# Autodesk Inventor assembly: unitychan
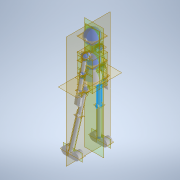
[picture p0: Inventor's stored thumbnail of the model, 180x180]
Saved by Autodesk Inventor 2021 (Build 250183000, 183)
## iProperties
Created: 2020-12-21
Part Number: unitychan
Document SubType Name: Assembly
Designer: Tazaki
Mass: 32000 g
Surface Area: 16434.1 cm^2
Volume: 27345.8 cm^3
Density: 1.1702 g/cm^3
Author: Tazaki
## Documents named in this file (19)
- C:\usr\Develop\choreonoid\BipedCnoid\model\unitychan\unitychan.iam
- C:\usr\Develop\choreonoid\BipedCnoid\model\unitychan\Hips.ipt
- C:\usr\Develop\choreonoid\BipedCnoid\model\unitychan\ChestY.ipt
- C:\usr\Develop\choreonoid\BipedCnoid\model\unitychan\ChestP.ipt
- C:\usr\Develop\choreonoid\BipedCnoid\model\unitychan\HeadY.ipt
- C:\usr\Develop\choreonoid\BipedCnoid\model\unitychan\HeadP.ipt
- C:\usr\Develop\choreonoid\BipedCnoid\model\unitychan\UpperarmP.ipt
- C:\usr\Develop\choreonoid\BipedCnoid\model\unitychan\UpperarmR.ipt
- C:\usr\Develop\choreonoid\BipedCnoid\model\unitychan\UpperarmY.ipt
- C:\usr\Develop\choreonoid\BipedCnoid\model\unitychan\LowerarmP.ipt
- C:\usr\Develop\choreonoid\BipedCnoid\model\unitychan\LowerarmY.ipt
- C:\usr\Develop\choreonoid\BipedCnoid\model\unitychan\HandP.ipt
- C:\usr\Develop\choreonoid\BipedCnoid\model\unitychan\HandY.ipt
- C:\usr\Develop\choreonoid\BipedCnoid\model\unitychan\UpperlegY.ipt
- C:\usr\Develop\choreonoid\BipedCnoid\model\unitychan\UpperlegR.ipt
- C:\usr\Develop\choreonoid\BipedCnoid\model\unitychan\UpperlegP.ipt
- C:\usr\Develop\choreonoid\BipedCnoid\model\unitychan\LowerlegP.ipt
- C:\usr\Develop\choreonoid\BipedCnoid\model\unitychan\FootR.ipt
- C:\usr\Develop\choreonoid\BipedCnoid\model\unitychan\FootP.ipt
## Components (31 placed, 18 different names)
1. Hips:1 — フラッシュ:1, フラッシュ:2, フラッシュ:3, メイト:1, フラッシュ:4, フラッシュ:21, メイト:18, フラッシュ:36, メイト:35
2. ChestY:1 — メイト:1, フラッシュ:4, メイト:2, フラッシュ:5
3. ChestP:1 — メイト:2, フラッシュ:5, メイト:3, フラッシュ:6, フラッシュ:27, メイト:24, メイト:27, メイト:28
4. HeadY:1 — メイト:3, フラッシュ:6, メイト:4, フラッシュ:7
5. HeadP:1 — メイト:4, フラッシュ:7
6. UpperarmP:1 — メイト:27, メイト:28, フラッシュ:30, メイト:29
7. UpperarmR:1 — フラッシュ:30, メイト:29, フラッシュ:31, メイト:30
8. UpperarmY:1 — フラッシュ:31, メイト:30, メイト:31, フラッシュ:32
9. LowerarmP:1 — メイト:31, フラッシュ:32, フラッシュ:33, メイト:32
10. LowerarmY:1 — フラッシュ:33, メイト:32, フラッシュ:34, メイト:33
11. HandP:1 — フラッシュ:34, メイト:33, フラッシュ:35, メイト:34
12. HandY:1 — フラッシュ:35, メイト:34
13. UpperlegY:1 — フラッシュ:36, メイト:35, フラッシュ:37, メイト:36
14. UpperlegR:1 — フラッシュ:37, メイト:36, フラッシュ:38, メイト:37
15. UpperlegP:1 — フラッシュ:38, メイト:37, フラッシュ:39, メイト:38
16. LowerlegP:1 — フラッシュ:39, メイト:38, フラッシュ:40, メイト:39
17. FootR:1 — フラッシュ:40, メイト:39, フラッシュ:41, メイト:40
18. FootP:1 — フラッシュ:41, メイト:40
19. UpperlegY:2 — フラッシュ:21, メイト:18, フラッシュ:22, メイト:19
20. UpperlegR:2 — フラッシュ:22, メイト:19, フラッシュ:23, メイト:20
21. UpperlegP:2 — フラッシュ:23, メイト:20, フラッシュ:24, メイト:21
22. LowerlegP:2 — フラッシュ:24, メイト:21, フラッシュ:25, メイト:22
23. FootP:2 — フラッシュ:26, メイト:23
24. FootR:2 — フラッシュ:25, メイト:22, フラッシュ:26, メイト:23
25. UpperarmP:2 — フラッシュ:27, メイト:24, フラッシュ:42, メイト:41
26. UpperarmY:2 — フラッシュ:43, メイト:42, フラッシュ:44, メイト:43
27. LowerarmP:2 — フラッシュ:44, メイト:43, フラッシュ:45, メイト:44
28. LowerarmY:2 — フラッシュ:45, メイト:44, フラッシュ:46, メイト:45
29. HandP:2 — フラッシュ:46, メイト:45, フラッシュ:47, メイト:46
30. HandY:2 — フラッシュ:47, メイト:46
31. UpperarmR:2 — フラッシュ:42, メイト:41, フラッシュ:43, メイト:42
## Relationships (63: Flush 32, Mate 31)
- フラッシュ:1 [Flush]: Hips:1
- フラッシュ:2 [Flush]: Hips:1
- フラッシュ:3 [Flush]: Hips:1
- メイト:1 [Mate]: Hips:1 ↔ ChestY:1
- フラッシュ:4 [Flush]: Hips:1 ↔ ChestY:1
- メイト:2 [Mate]: ChestY:1 ↔ ChestP:1
- フラッシュ:5 [Flush]: ChestY:1 ↔ ChestP:1
- メイト:3 [Mate]: ChestP:1 ↔ HeadY:1
- フラッシュ:6 [Flush]: ChestP:1 ↔ HeadY:1
- メイト:4 [Mate]: HeadY:1 ↔ HeadP:1
- フラッシュ:7 [Flush]: HeadY:1 ↔ HeadP:1
- フラッシュ:21 [Flush]: Hips:1 ↔ UpperlegY:2
- メイト:18 [Mate]: Hips:1 ↔ UpperlegY:2
- フラッシュ:22 [Flush]: UpperlegY:2 ↔ UpperlegR:2
- メイト:19 [Mate]: UpperlegY:2 ↔ UpperlegR:2
- フラッシュ:23 [Flush]: UpperlegR:2 ↔ UpperlegP:2
- メイト:20 [Mate]: UpperlegR:2 ↔ UpperlegP:2
- フラッシュ:24 [Flush]: UpperlegP:2 ↔ LowerlegP:2
- メイト:21 [Mate]: UpperlegP:2 ↔ LowerlegP:2
- フラッシュ:25 [Flush]: LowerlegP:2 ↔ FootR:2
- メイト:22 [Mate]: LowerlegP:2 ↔ FootR:2
- フラッシュ:26 [Flush]: FootP:2 ↔ FootR:2
- メイト:23 [Mate]: FootP:2 ↔ FootR:2
- フラッシュ:27 [Flush]: ChestP:1 ↔ UpperarmP:2
- メイト:24 [Mate]: ChestP:1 ↔ UpperarmP:2
- メイト:27 [Mate]: ChestP:1 ↔ UpperarmP:1
- メイト:28 [Mate]: ChestP:1 ↔ UpperarmP:1
- フラッシュ:30 [Flush]: UpperarmP:1 ↔ UpperarmR:1
- メイト:29 [Mate]: UpperarmP:1 ↔ UpperarmR:1
- フラッシュ:31 [Flush]: UpperarmR:1 ↔ UpperarmY:1
- メイト:30 [Mate]: UpperarmR:1 ↔ UpperarmY:1
- メイト:31 [Mate]: UpperarmY:1 ↔ LowerarmP:1
- フラッシュ:32 [Flush]: UpperarmY:1 ↔ LowerarmP:1
- フラッシュ:33 [Flush]: LowerarmP:1 ↔ LowerarmY:1
- メイト:32 [Mate]: LowerarmP:1 ↔ LowerarmY:1
- フラッシュ:34 [Flush]: LowerarmY:1 ↔ HandP:1
- メイト:33 [Mate]: LowerarmY:1 ↔ HandP:1
- フラッシュ:35 [Flush]: HandP:1 ↔ HandY:1
- メイト:34 [Mate]: HandP:1 ↔ HandY:1
- フラッシュ:36 [Flush]: Hips:1 ↔ UpperlegY:1
- メイト:35 [Mate]: Hips:1 ↔ UpperlegY:1
- フラッシュ:37 [Flush]: UpperlegY:1 ↔ UpperlegR:1
- メイト:36 [Mate]: UpperlegY:1 ↔ UpperlegR:1
- フラッシュ:38 [Flush]: UpperlegR:1 ↔ UpperlegP:1
- メイト:37 [Mate]: UpperlegR:1 ↔ UpperlegP:1
- フラッシュ:39 [Flush]: UpperlegP:1 ↔ LowerlegP:1
- メイト:38 [Mate]: UpperlegP:1 ↔ LowerlegP:1
- フラッシュ:40 [Flush]: LowerlegP:1 ↔ FootR:1
- メイト:39 [Mate]: LowerlegP:1 ↔ FootR:1
- フラッシュ:41 [Flush]: FootR:1 ↔ FootP:1
- メイト:40 [Mate]: FootR:1 ↔ FootP:1
- フラッシュ:42 [Flush]: UpperarmP:2 ↔ UpperarmR:2
- メイト:41 [Mate]: UpperarmP:2 ↔ UpperarmR:2
- フラッシュ:43 [Flush]: UpperarmY:2 ↔ UpperarmR:2
- メイト:42 [Mate]: UpperarmY:2 ↔ UpperarmR:2
- フラッシュ:44 [Flush]: UpperarmY:2 ↔ LowerarmP:2
- メイト:43 [Mate]: UpperarmY:2 ↔ LowerarmP:2
- フラッシュ:45 [Flush]: LowerarmP:2 ↔ LowerarmY:2
- メイト:44 [Mate]: LowerarmP:2 ↔ LowerarmY:2
- フラッシュ:46 [Flush]: LowerarmY:2 ↔ HandP:2
- メイト:45 [Mate]: LowerarmY:2 ↔ HandP:2
- フラッシュ:47 [Flush]: HandP:2 ↔ HandY:2
- メイト:46 [Mate]: HandP:2 ↔ HandY:2
